# Autodesk Inventor assembly: E001-Chambre
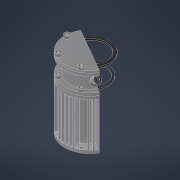
[picture p0: Inventor's stored thumbnail of the model, 180x180]
Saved by Autodesk Inventor 2021.3 (Build 253353000, 353)
## iProperties
Company: HES-SO
Created: 2022-03-31
Part Number: E001-Chambre
Document SubType Name: Assembly
Designer: HER & ZAE
Author: HER & ZAE
## Documents named in this file (16)
- C:\Users\remi\OneDrive\Documents\Cours\05-HEVS\S2fb\mechanic\CCo\project\Compressor\E001-Chambre.iam
- C:\Users\remi\OneDrive\Documents\Cours\05-HEVS\S2fb\mechanic\CCo\project\Compressor\P002-Bati_chambre.ipt
- C:\Users\remi\OneDrive\Documents\Cours\05-HEVS\S2fb\mechanic\CCo\project\Compressor\P001-Couverture.ipt
- C:\Users\remi\OneDrive\Documents\Cours\05-HEVS\S2fb\mechanic\CCo\project\Compressor\P011-Chapeau_chambre.ipt
- C:\Users\remi\OneDrive\Documents\Cours\05-HEVS\S2fb\mechanic\CCo\project\Compressor\E001-Chambre\Design Accelerator\O-Ring3.iam
- C:\Users\remi\OneDrive\Documents\Cours\05-HEVS\S2fb\mechanic\CCo\project\Compressor\R2021\en-US\AS 1420\AS 1420 - 1973 - M3 x 6.ipt
- C:\Users\remi\OneDrive\Documents\Cours\05-HEVS\S2fb\mechanic\CCo\project\Compressor\P006-Soupape\P006-Soupape_IN.ipt
- C:\Users\remi\OneDrive\Documents\Cours\05-HEVS\S2fb\mechanic\CCo\project\Compressor\P006-Soupape.ipt
- C:\Users\remi\OneDrive\Documents\Cours\05-HEVS\S2fb\mechanic\CCo\project\Compressor\P006-Soupape\P006-Soupape_OUT.ipt
- C:\Users\remi\OneDrive\Documents\Cours\05-HEVS\S2fb\mechanic\CCo\project\Compressor\P019-Chapeau_tete_chambre.ipt
- C:\Users\remi\OneDrive\Documents\Cours\05-HEVS\S2fb\mechanic\CCo\project\Compressor\E001-Chambre\Design Accelerator\O-Ring4.iam
- C:\Users\remi\OneDrive\Documents\Cours\05-HEVS\S2fb\mechanic\CCo\project\Compressor\E001-Chambre\Design Accelerator\O-Ring8.iam
- C:\Users\remi\OneDrive\Documents\Cours\05-HEVS\S2fb\mechanic\CCo\project\Compressor\E001-Chambre\Design Accelerator\O-Ring6.iam
- C:\Users\remi\OneDrive\Documents\Cours\05-HEVS\S2fb\mechanic\CCo\project\Compressor\Circlips\ungespannt_61799403.ipt
- C:\Users\remi\OneDrive\Documents\Cours\05-HEVS\S2fb\mechanic\CCo\project\Compressor\Compress Spring14.ipt
- C:\Users\remi\OneDrive\Documents\Cours\05-HEVS\S2fb\mechanic\CCo\project\Compressor\Compress Spring15.ipt
## Components (25 placed, 10 different names)
1. P002-Bati_chambre:1 — Mate:1, Flush:1, Mate:3, Mate:4, Mate:5
2. P001-Couverture:1 — Mate:1, Flush:1, Mate:2
3. P011-Chapeau_chambre:1 — Mate:2, Mate:3, Mate:6, Mate:7, Mate:8, Mate:9, Mate:10, Mate:11, Mate:12, Mate:13, Mate:14, Mate:15, Mate:16, Mate:17, Mate:20, Mate:21, Mate:22, Mate:23, Mate:24, Mate:27, Flush:2, Mate:30, Mate:31, Mate:32, Flush:4, Flush:6
4. O-Ring:1 [sub-assembly] — Mate:4, Mate:5
5. P006-Soupape_OUT:1 — Flush:2, Mate:35, Mate:36
6. P006-Soupape_IN:2 — Mate:32, Flush:4, Mate:33, Mate:34, Mate:37
7. P019-Chapeau_tete_chambre:1 — Mate:20, Mate:21, Mate:22, Insert:1, Insert:2, Insert:3, Insert:4, Insert:5, Insert:6, Mate:27, Flush:5, Mate:36
8. O-Ring:2 [sub-assembly] — Mate:23, Mate:24
9. O-Ring:3 [sub-assembly] — Mate:30
10. O-Ring:4 [sub-assembly] — Mate:31
11. ungespannt_61799403:1 — Mate:33, Mate:34
12. Compress Spring1:1 — Mate:35, Flush:5
13. Compress Spring1:1 — Mate:37, Flush:6
14. AS 1420 - Metric M3 x 6:7 — Insert:1
15. AS 1420 - Metric M3 x 6:8 — Insert:2
16. AS 1420 - Metric M3 x 6:9 — Insert:3
17. AS 1420 - Metric M3 x 6:10 — Insert:4
18. AS 1420 - Metric M3 x 6:11 — Insert:5
19. AS 1420 - Metric M3 x 6:12 — Insert:6
20. AS 1420 - Metric M3 x 6:1 — Mate:6, Mate:7
21. AS 1420 - Metric M3 x 6:2 — Mate:8, Mate:9
22. AS 1420 - Metric M3 x 6:3 — Mate:10, Mate:11
23. AS 1420 - Metric M3 x 6:4 — Mate:12, Mate:13
24. AS 1420 - Metric M3 x 6:5 — Mate:14, Mate:15
25. AS 1420 - Metric M3 x 6:6 — Mate:16, Mate:17
## Relationships (42: Mate 31, Insert 6, Flush 5)
- Mate:1: P002-Bati_chambre:1 ↔ P001-Couverture:1
- Flush:1: P002-Bati_chambre:1 ↔ P001-Couverture:1
- Mate:2: P001-Couverture:1 ↔ P011-Chapeau_chambre:1
- Mate:3: P002-Bati_chambre:1 ↔ P011-Chapeau_chambre:1
- Mate:4: P002-Bati_chambre:1 ↔ O-Ring:1
- Mate:5: P002-Bati_chambre:1 ↔ O-Ring:1
- Mate:6: P011-Chapeau_chambre:1 ↔ AS 1420 - Metric M3 x 6:1
- Mate:7: P011-Chapeau_chambre:1 ↔ AS 1420 - Metric M3 x 6:1
- Mate:8: P011-Chapeau_chambre:1 ↔ AS 1420 - Metric M3 x 6:2
- Mate:9: P011-Chapeau_chambre:1 ↔ AS 1420 - Metric M3 x 6:2
- Mate:10: P011-Chapeau_chambre:1 ↔ AS 1420 - Metric M3 x 6:3
- Mate:11: P011-Chapeau_chambre:1 ↔ AS 1420 - Metric M3 x 6:3
- Mate:12: P011-Chapeau_chambre:1 ↔ AS 1420 - Metric M3 x 6:4
- Mate:13: P011-Chapeau_chambre:1 ↔ AS 1420 - Metric M3 x 6:4
- Mate:14: P011-Chapeau_chambre:1 ↔ AS 1420 - Metric M3 x 6:5
- Mate:15: P011-Chapeau_chambre:1 ↔ AS 1420 - Metric M3 x 6:5
- Mate:16: P011-Chapeau_chambre:1 ↔ AS 1420 - Metric M3 x 6:6
- Mate:17: P011-Chapeau_chambre:1 ↔ AS 1420 - Metric M3 x 6:6
- Mate:20: P011-Chapeau_chambre:1 ↔ P019-Chapeau_tete_chambre:1
- Mate:21: P011-Chapeau_chambre:1 ↔ P019-Chapeau_tete_chambre:1
- Mate:22: P011-Chapeau_chambre:1 ↔ P019-Chapeau_tete_chambre:1
- Mate:23: P011-Chapeau_chambre:1 ↔ O-Ring:2
- Mate:24: P011-Chapeau_chambre:1 ↔ O-Ring:2
- Insert:1: P019-Chapeau_tete_chambre:1 ↔ AS 1420 - Metric M3 x 6:7
- Insert:2: P019-Chapeau_tete_chambre:1 ↔ AS 1420 - Metric M3 x 6:8
- Insert:3: P019-Chapeau_tete_chambre:1 ↔ AS 1420 - Metric M3 x 6:9
- Insert:4: P019-Chapeau_tete_chambre:1 ↔ AS 1420 - Metric M3 x 6:10
- Insert:5: P019-Chapeau_tete_chambre:1 ↔ AS 1420 - Metric M3 x 6:11
- Insert:6: P019-Chapeau_tete_chambre:1 ↔ AS 1420 - Metric M3 x 6:12
- Mate:27: P011-Chapeau_chambre:1 ↔ P019-Chapeau_tete_chambre:1
- Flush:2 (1 mm): P011-Chapeau_chambre:1 ↔ P006-Soupape_OUT:1
- Mate:30: P011-Chapeau_chambre:1 ↔ O-Ring:3
- Mate:31: P011-Chapeau_chambre:1 ↔ O-Ring:4
- Mate:32: P011-Chapeau_chambre:1 ↔ P006-Soupape_IN:2
- Flush:4: P011-Chapeau_chambre:1 ↔ P006-Soupape_IN:2
- Mate:33: P006-Soupape_IN:2 ↔ ungespannt_61799403:1
- Mate:34: P006-Soupape_IN:2 ↔ ungespannt_61799403:1
- Mate:35: P006-Soupape_OUT:1 ↔ Compress Spring1:1
- Flush:5: P019-Chapeau_tete_chambre:1 ↔ Compress Spring1:1
- Mate:36: P006-Soupape_OUT:1 ↔ P019-Chapeau_tete_chambre:1
- Mate:37: P006-Soupape_IN:2 ↔ Compress Spring1:1
- Flush:6: P011-Chapeau_chambre:1 ↔ Compress Spring1:1
